# Autodesk Inventor assembly: Horizontal Weapon Assembly (Type Spd)
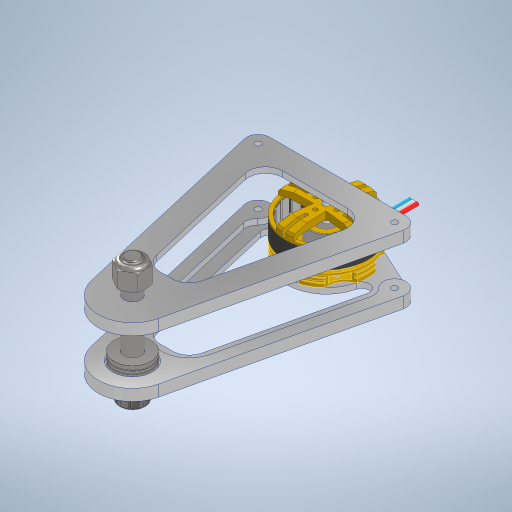
[picture p0: Inventor's stored thumbnail of the model, 512x512]
Saved by Autodesk Inventor 2023.2 (Build 272271000, 271)
## iProperties
Created: 2023-03-06
Part Number: Horizontal Weapon Assembly (Type Spd)
Document SubType Name: Assembly
Designer: Nathan Cai
Author: Nathan Cai
## Documents named in this file (7)
- C:\Users\Nathan Cai\Documents\Inventor\0.3rd Lawette - V3.6\Horizontal Weapon Assembly (Type Spd)\Horizontal Weapon Assembly (Type Spd).iam
- C:\Users\Nathan Cai\Documents\Inventor\0.3rd Lawette - V3.6\Horizontal Weapon Assembly (Type Spd)\Frame (Clear Side).ipt
- C:\Users\Nathan Cai\Documents\Inventor\0.3rd Lawette - V3.6\Horizontal Weapon Assembly (Type Spd)\Frame (Motor Side).ipt
- C:\Users\Nathan Cai\Documents\Inventor\0.3rd Lawette - V3.6\Horizontal Weapon Assembly (Type Spd)\90807A139_Same-Size Thread Alloy Steel Shoulder Screw.ipt
- C:\Users\Nathan Cai\Documents\Inventor\0.3rd Lawette - V3.6\Horizontal Weapon Assembly (Type Spd)\90630A121_High-Strength Steel Nylon-Insert Locknut.ipt
- C:\Users\Nathan Cai\Documents\Inventor\0.3rd Lawette - V3.6\Horizontal Weapon Assembly (Type Spd)\Thrust Ball Bearing.ipt
- C:\Users\Nathan Cai\Documents\Inventor\0.3rd Lawette - V3.6\FEICHAO BE4108 380KV\FEICHAO BE4108 380KV.iam
## Components (7 placed, 6 different names)
1. Frame (Motor Side):1 — Mate:1, Mate:2, Mate:3, Mate:7, Mate:8, Mate:12, Mate:13, Mate:14
2. Frame (Clear Side):1 — Mate:1, Mate:2, Mate:3, Mate:6, Mate:10
3. 90807A139_Same-Size Thread Alloy Steel Shoulder Screw:1 — Mate:4, Mate:5, Mate:6, Mate:7, Mate:9, Mate:11
4. 90630A121_High-Strength Steel Nylon-Insert Locknut:1 — Mate:4, Mate:5
5. Thrust Ball Bearing:1 — Mate:8, Mate:9
6. Thrust Ball Bearing:2 — Mate:10, Mate:11
7. FEICHAO BE4108 380KV:1 [sub-assembly] — Mate:12, Mate:13, Mate:14
## Relationships (14: Mate 14)
- Mate:1: Frame (Motor Side):1 ↔ Frame (Clear Side):1
- Mate:2 (25.4 mm): Frame (Motor Side):1 ↔ Frame (Clear Side):1
- Mate:3: Frame (Motor Side):1 ↔ Frame (Clear Side):1
- Mate:4: 90807A139_Same-Size Thread Alloy Steel Shoulder Screw:1 ↔ 90630A121_High-Strength Steel Nylon-Insert Locknut:1
- Mate:5: 90807A139_Same-Size Thread Alloy Steel Shoulder Screw:1 ↔ 90630A121_High-Strength Steel Nylon-Insert Locknut:1
- Mate:6: Frame (Clear Side):1 ↔ 90807A139_Same-Size Thread Alloy Steel Shoulder Screw:1
- Mate:7 (6.35 mm): Frame (Motor Side):1 ↔ 90807A139_Same-Size Thread Alloy Steel Shoulder Screw:1
- Mate:8 (0.0254 mm): Frame (Motor Side):1 ↔ Thrust Ball Bearing:1
- Mate:9: 90807A139_Same-Size Thread Alloy Steel Shoulder Screw:1 ↔ Thrust Ball Bearing:1
- Mate:10 (0.0254 mm): Frame (Clear Side):1 ↔ Thrust Ball Bearing:2
- Mate:11: 90807A139_Same-Size Thread Alloy Steel Shoulder Screw:1 ↔ Thrust Ball Bearing:2
- Mate:12: Frame (Motor Side):1 ↔ FEICHAO BE4108 380KV:1
- Mate:13: Frame (Motor Side):1 ↔ FEICHAO BE4108 380KV:1
- Mate:14: Frame (Motor Side):1 ↔ FEICHAO BE4108 380KV:1
